# Autodesk Inventor assembly: chassis
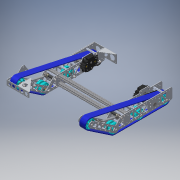
[picture p0: Inventor's stored thumbnail of the model, 180x180]
Saved by Autodesk Inventor 2019 (Build 230136000, 136)
## iProperties
Created: 2016-01-20
Part Number: chassis
Description: STEP AP214
Document SubType Name: Assembly
Designer: Spooner
Sending System: SolidWorks 2014
Preprocessor: SwSTEP 2.0
Title: am-3358 Bumper Kit for Rhino Track Drive Module.STEP
Revision Number: ANY
## Documents named in this file (6)
- C:\Users\Student\Documents\Inventor\2019 Chassis\chassis.iam
- C:\Users\Student\Documents\Inventor\2019 Chassis\STEP Files\am-3352 Rhino Front Left Bumper Bracket.ipt
- C:\Users\Student\Documents\Inventor\2019 Chassis\STEP Files\am-3354 Rhino Back Left Bumper Bracket.ipt
- C:\Users\Student\Documents\Inventor\2019 Chassis\STEP Files\am-3322 Rhino Track Drive Module Left.iam
- C:\Users\Student\Documents\Inventor\2019 Chassis\STEP Files\am-3322 Rhino Track Drive Module Right.iam
- C:\Users\Student\Documents\Inventor\2019 Chassis\27inch - 47065T977_ALUMINUM T-SLOTTED FRAMING EXTRUSION.ipt
## Components (6 placed, 5 different names)
1. am-3322 Rhino Track Drive Module Left:1 [sub-assembly] — Flush:1, Flush:2, Flush:3, Mate:7
2. am-3322 Rhino Track Drive Module Right:1 [sub-assembly] — Flush:1, Flush:2, Flush:3, Mate:2, Mate:3, Angle:1, Mate:4, Mate:5, Angle:2, Mate:6, Angle:3, Mate:8, Mate:9, Mate:10
3. am-3354 Rhino Back Left Bumper Bracket:1 — Mate:4, Mate:5, Angle:2
4. am-3352 Rhino Front Left Bumper Bracket:1 — Mate:2, Mate:3, Angle:1
5. 27inch - 47065T977_ALUMINUM T-SLOTTED FRAMING EXTRUSION:1 — Mate:6, Angle:3, Mate:7, Mate:8, Angle:4
6. 27inch - 47065T977_ALUMINUM T-SLOTTED FRAMING EXTRUSION:2 — Mate:9, Mate:10, Angle:4
## Relationships (16: Mate 9, Angle 4, Flush 3)
- Flush:1: am-3322 Rhino Track Drive Module Left:1 ↔ am-3322 Rhino Track Drive Module Right:1
- Flush:2: am-3322 Rhino Track Drive Module Left:1 ↔ am-3322 Rhino Track Drive Module Right:1
- Flush:3: am-3322 Rhino Track Drive Module Left:1 ↔ am-3322 Rhino Track Drive Module Right:1
- Mate:2: am-3322 Rhino Track Drive Module Right:1 ↔ am-3352 Rhino Front Left Bumper Bracket:1
- Mate:3: am-3322 Rhino Track Drive Module Right:1 ↔ am-3352 Rhino Front Left Bumper Bracket:1
- Angle:1 (0 deg): am-3322 Rhino Track Drive Module Right:1 ↔ am-3352 Rhino Front Left Bumper Bracket:1
- Mate:4: am-3322 Rhino Track Drive Module Right:1 ↔ am-3354 Rhino Back Left Bumper Bracket:1
- Mate:5: am-3322 Rhino Track Drive Module Right:1 ↔ am-3354 Rhino Back Left Bumper Bracket:1
- Angle:2 (0 deg): am-3322 Rhino Track Drive Module Right:1 ↔ am-3354 Rhino Back Left Bumper Bracket:1
- Mate:6: am-3322 Rhino Track Drive Module Right:1 ↔ 27inch - 47065T977_ALUMINUM T-SLOTTED FRAMING EXTRUSION:1
- Angle:3 (0 deg): am-3322 Rhino Track Drive Module Right:1 ↔ 27inch - 47065T977_ALUMINUM T-SLOTTED FRAMING EXTRUSION:1
- Mate:7: am-3322 Rhino Track Drive Module Left:1 ↔ 27inch - 47065T977_ALUMINUM T-SLOTTED FRAMING EXTRUSION:1
- Mate:8: am-3322 Rhino Track Drive Module Right:1 ↔ 27inch - 47065T977_ALUMINUM T-SLOTTED FRAMING EXTRUSION:1
- Mate:9: am-3322 Rhino Track Drive Module Right:1 ↔ 27inch - 47065T977_ALUMINUM T-SLOTTED FRAMING EXTRUSION:2
- Mate:10: am-3322 Rhino Track Drive Module Right:1 ↔ 27inch - 47065T977_ALUMINUM T-SLOTTED FRAMING EXTRUSION:2
- Angle:4 (0 deg): 27inch - 47065T977_ALUMINUM T-SLOTTED FRAMING EXTRUSION:1 ↔ 27inch - 47065T977_ALUMINUM T-SLOTTED FRAMING EXTRUSION:2
